# Autodesk Inventor assembly: heatsink
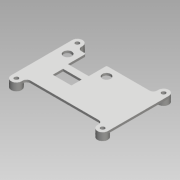
[picture p0: Inventor's stored thumbnail of the model, 180x180]
Saved by Autodesk Inventor 2018 (Build 220112000, 112)
## iProperties
Created: 2019-09-11
Part Number: heatsink
Document SubType Name: Assembly
Designer: vfv13
Author: vfv13
## iProperties of the stored document COMPOUND_2.ipt
Created: 2019-09-11
Part Number: COMPOUND_2
Material: Generic
Document SubType Name: Modeling
Designer: vfv13
Density: 1 g/cm^3
Appearance: Default
Author: vfv13
## iProperties of the stored document SOLID_4.ipt
Created: 2019-09-11
Part Number: SOLID_4
Material: Generic
Document SubType Name: Modeling
Designer: vfv13
Density: 1 g/cm^3
Appearance: Default
Author: vfv13
## iProperties of the stored document JST_XH_B4B-XH-A_1x04_P2.50mm_Vertical.iam
Created: 2019-09-11
Part Number: JST_XH_B4B-XH-A_1x04_P2.50mm_Vertical
Document SubType Name: Assembly
Designer: vfv13
Author: vfv13
## iProperties of the stored document BQ76200PWR.iam
Created: 2019-09-11
Part Number: BQ76200PWR
Document SubType Name: Assembly
Designer: vfv13
Author: vfv13
## iProperties of the stored document COMPOUND.ipt
Created: 2019-09-11
Part Number: COMPOUND
Material: Generic
Document SubType Name: Modeling
Designer: vfv13
Density: 1 g/cm^3
Appearance: Default
Author: vfv13
## iProperties of the stored document Anti-Spark.iam
Company: A Company
Created: 2019-09-11
Part Number: Anti-Spark
Description: KiCad electronic assembly
Document SubType Name: Assembly
Designer: vfv13
Authority: Unknown
Title: Anti-Spark.step
Author: An Author
Sending System: KiCad to STEP converter
Preprocessor: Open CASCADE STEP processor 6.9
## iProperties of the stored document COMPOUND_1.ipt
Created: 2019-09-11
Part Number: COMPOUND_1
Material: Generic
Document SubType Name: Modeling
Designer: vfv13
Density: 1 g/cm^3
Appearance: Default
Author: vfv13
## iProperties of the stored document TPS7A4101DGNR.iam
Created: 2019-09-11
Part Number: TPS7A4101DGNR
Document SubType Name: Assembly
Designer: vfv13
Author: vfv13
## iProperties of the stored document SOLID_1.ipt
Created: 2019-09-11
Part Number: SOLID_1
Material: Generic
Document SubType Name: Modeling
Designer: vfv13
Density: 1 g/cm^3
Appearance: Default
Author: vfv13
## iProperties of the stored document C_0805_2012Metric.iam
Created: 2019-09-11
Part Number: C_0805_2012Metric
Document SubType Name: Assembly
Designer: vfv13
Author: vfv13
## iProperties of the stored document SOT1215.iam
Created: 2019-09-11
Part Number: SOT1215
Document SubType Name: Assembly
Designer: vfv13
Author: vfv13
## iProperties of the stored document SOLID_3.ipt
Created: 2019-09-11
Part Number: SOLID_3
Material: Generic
Document SubType Name: Modeling
Designer: vfv13
Density: 1 g/cm^3
Appearance: Default
Author: vfv13
## iProperties of the stored document D_SOD-323.iam
Created: 2019-09-11
Part Number: D_SOD-323
Document SubType Name: Assembly
Designer: vfv13
Author: vfv13
## iProperties of the stored document SOLID.ipt
Created: 2019-09-11
Part Number: SOLID
Material: Generic
Document SubType Name: Modeling
Designer: vfv13
Density: 1 g/cm^3
Appearance: Default
Author: vfv13
## iProperties of the stored document R_0805_2012Metric.iam
Created: 2019-09-11
Part Number: R_0805_2012Metric
Document SubType Name: Assembly
Designer: vfv13
Author: vfv13
## iProperties of the stored document SOLID_2.ipt
Created: 2019-09-11
Part Number: SOLID_2
Material: Generic
Document SubType Name: Modeling
Designer: vfv13
Density: 1 g/cm^3
Appearance: Default
Author: vfv13
## Documents named in this file (20)
- D:\Dokumente\Elektronik\Mountainboard\Anti-Spark\Anti-Spark\High-Side-NMOS-Antispark-Switch\heatsink.iam
- **D:\Dokumente\Elektronik\Mountainboard\Anti-Spark\Anti-Spark\High-Side-NMOS-Antispark-Switch\heatsink.iam*LocalDocs*x50oq421pFdxoup4gH3rv02hoRg*Anti-Spark.iam
- D:\Dokumente\3D Drucker\tischerhöhung\Part18.ipt
- D:\Dokumente\3D Drucker\tischerhöhung\heatsink.ipt
- **D:\Dokumente\Elektronik\Mountainboard\Anti-Spark\Anti-Spark\High-Side-NMOS-Antispark-Switch\heatsink.iam*LocalDocs*xTbkhrnw1Tvdvemca4izcxnrtZh*COMPOUND_2.ipt
- **D:\Dokumente\Elektronik\Mountainboard\Anti-Spark\Anti-Spark\High-Side-NMOS-Antispark-Switch\heatsink.iam*LocalDocs*xDqoj44vsQ02getkkP42jpcrrKb*SOLID_4.ipt
- **D:\Dokumente\Elektronik\Mountainboard\Anti-Spark\Anti-Spark\High-Side-NMOS-Antispark-Switch\heatsink.iam*LocalDocs*xD1ga2wm52amuuwoy4zvrat0d5h*JST_XH_B4B-XH-A_1x04_P2.50mm_Vertical.iam
- **D:\Dokumente\Elektronik\Mountainboard\Anti-Spark\Anti-Spark\High-Side-NMOS-Antispark-Switch\heatsink.iam*LocalDocs*xHwtto2ztRivwu14aDeyujr2j2g*SOLID_1.ipt
- **D:\Dokumente\Elektronik\Mountainboard\Anti-Spark\Anti-Spark\High-Side-NMOS-Antispark-Switch\heatsink.iam*LocalDocs*x4uvhvr01Rdtie1kuWsbypiorVc*BQ76200PWR.iam
- **D:\Dokumente\Elektronik\Mountainboard\Anti-Spark\Anti-Spark\High-Side-NMOS-Antispark-Switch\heatsink.iam*LocalDocs*xD5hbrr1tKoasem02Eavkp5gqSe*COMPOUND_1.ipt
- **D:\Dokumente\Elektronik\Mountainboard\Anti-Spark\Anti-Spark\High-Side-NMOS-Antispark-Switch\heatsink.iam*LocalDocs*x0dohv51oNnxlev45S4dcwpvkXd*COMPOUND.ipt
- **D:\Dokumente\Elektronik\Mountainboard\Anti-Spark\Anti-Spark\High-Side-NMOS-Antispark-Switch\heatsink.iam*LocalDocs*xQjz5gweqLw2kuq4cLjqjozruUf*SOT1215.iam
- **D:\Dokumente\Elektronik\Mountainboard\Anti-Spark\Anti-Spark\High-Side-NMOS-Antispark-Switch\heatsink.iam*LocalDocs*xJpm355qjPrpyezocU03vmyebDd*TPS7A4101DGNR.iam
- **D:\Dokumente\Elektronik\Mountainboard\Anti-Spark\Anti-Spark\High-Side-NMOS-Antispark-Switch\heatsink.iam*LocalDocs*xQoolvjm2Xtkxem0yKpogjeh12g*C_0805_2012Metric.iam
- **D:\Dokumente\Elektronik\Mountainboard\Anti-Spark\Anti-Spark\High-Side-NMOS-Antispark-Switch\heatsink.iam*LocalDocs*xZmmlrwxuHhrveoo0Yyvtm4wdCa*R_0805_2012Metric.iam
- **D:\Dokumente\Elektronik\Mountainboard\Anti-Spark\Anti-Spark\High-Side-NMOS-Antispark-Switch\heatsink.iam*LocalDocs*xYypvviuvNjr1etgwKdfikp5kNh*D_SOD-323.iam
- **D:\Dokumente\Elektronik\Mountainboard\Anti-Spark\Anti-Spark\High-Side-NMOS-Antispark-Switch\heatsink.iam*LocalDocs*xZgn1vfdeItz5u3giJrda3olx0h*SOLID_2.ipt
- **D:\Dokumente\Elektronik\Mountainboard\Anti-Spark\Anti-Spark\High-Side-NMOS-Antispark-Switch\heatsink.iam*LocalDocs*xTrsaa3ktP4unuwgcXv35gkt3Sc*SOLID.ipt
- **D:\Dokumente\Elektronik\Mountainboard\Anti-Spark\Anti-Spark\High-Side-NMOS-Antispark-Switch\heatsink.iam*LocalDocs*xZ5yziiryZwlaezw5Ksdud2gkWb*SOLID_3.ipt
- D:\Dokumente\Elektronik\Mountainboard\Anti-Spark\Anti-Spark\High-Side-NMOS-Antispark-Switch\Anti-Spark.step
## Components (3 placed, 3 different names)
1. Anti-Spark:1 [sub-assembly] — Flush:1, Flush:6, Flush:7, Flush:8, Flush:9
2. Part18:1 — Flush:1, Flush:6, Flush:7
3. heatsink:1 — Flush:8, Flush:9
## Relationships (5: Flush 5)
- Flush:1: Anti-Spark:1 ↔ Part18:1
- Flush:6: Anti-Spark:1 ↔ Part18:1
- Flush:7: Anti-Spark:1 ↔ Part18:1
- Flush:8: Anti-Spark:1 ↔ heatsink:1
- Flush:9: Anti-Spark:1 ↔ heatsink:1
